# Autodesk Inventor assembly: gu1e_round-round
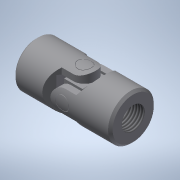
[picture p0: Inventor's stored thumbnail of the model, 180x180]
Saved by Autodesk Inventor 2021.2 (Build 252289000, 289)
## iProperties
Created: 2021-03-16
Part Number: gu1e_round-round
Checked By: TraceParts S.A.
Catalog Web Link: www.traceparts.com
Document SubType Name: Assembly
Designer: TraceParts
Company: TraceParts S.A.
DESIGN: GUE cardanic DIN808
SUPPLIER: SIT
TraceParts.PartNumber: 32-28022007-067680
TraceParts.PartTitle: GUE cardanic DIN808
TraceParts.InstanceId: 32-28022007-067680JHA2HX92DB50YX739C172EFG
TraceParts.PartStatus: Published
TraceParts.PartVersion: 1.1.7
TRACEPARTS: TRACEPARTS
TraceParts.PartLanguage: en
TraceParts.ClassPath: SIT:32-28022007-067680
Author: TraceParts
## Documents named in this file (4)
- C:\Users\equip\Documents\AAA Nacho Mecatrónica\Nacho Sexto Semestre MT\Diseño Mecatrónico\gu1e_round-round.iam
- C:\Users\equip\Documents\AAA Nacho Mecatrónica\Nacho Sexto Semestre MT\Diseño Mecatrónico\gu1e_round-round_01.ipt
- C:\Users\equip\Documents\AAA Nacho Mecatrónica\Nacho Sexto Semestre MT\Diseño Mecatrónico\gu1e_round-round_02.ipt
- C:\Users\equip\Documents\AAA Nacho Mecatrónica\Nacho Sexto Semestre MT\Diseño Mecatrónico\gu1e_round-round_03.ipt
## Components (3 placed, 3 different names)
1. gu1e_round-round_01:1 — Insertar:2
2. gu1e_round-round_02:1 — Insertar:1
3. gu1e_round-round_03:1 — Insertar:1, Insertar:2
## Relationships (2: Insert 2)
- Insertar:1: gu1e_round-round_02:1 ↔ gu1e_round-round_03:1
- Insertar:2: gu1e_round-round_01:1 ↔ gu1e_round-round_03:1
